# Autodesk Inventor assembly: CorpoInternoTurbinaAssemblato
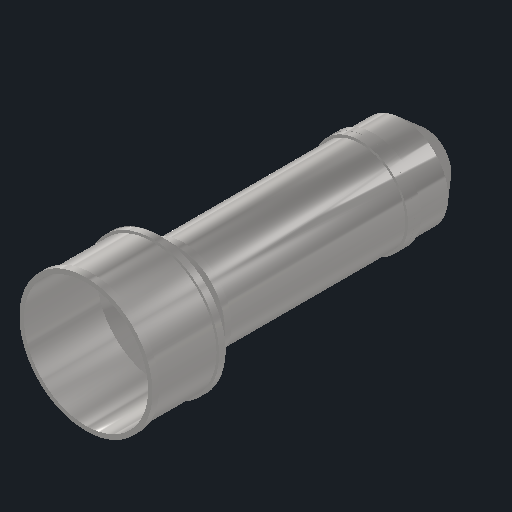
[picture p0: Inventor's stored thumbnail of the model, 512x512]
Saved by Autodesk Inventor 2026.2 (Build 302298010, 298A)
## iProperties
Created: 2026-05-01
Part Number: CorpoInternoTurbinaAssemblato
Document SubType Name: Assembly
Designer: Yan
Author: Yan
## Documents named in this file (5)
- C:\Users\Yan\Desktop\Turbina\CorpoInternoTurbinaAssemblato.iam
- C:\Users\Yan\Desktop\Turbina\CollegamentoCorpo1.ipt
- C:\Users\Yan\Desktop\Turbina\DiscoCorpoScarico.ipt
- C:\Users\Yan\Desktop\Turbina\DiscoCorpoTurbina2.ipt
- C:\Users\Yan\Desktop\Turbina\DiscoCorpoTurbina3.ipt
## Components (4 placed, 4 different names)
1. CollegamentoCorpo1:1 — Mate:1, Mate:2, Mate:4, Mate:5, Mate:6
2. DiscoCorpoScarico:1 — Mate:7, Mate:8
3. DiscoCorpoTurbina2:1 — Mate:1, Mate:3, Mate:4, Mate:6
4. DiscoCorpoTurbina3:1 — Mate:2, Mate:3, Mate:5, Mate:7, Mate:8
## Relationships (8: Mate 8)
- Mate:1: CollegamentoCorpo1:1 ↔ DiscoCorpoTurbina2:1
- Mate:2: CollegamentoCorpo1:1 ↔ DiscoCorpoTurbina3:1
- Mate:3: DiscoCorpoTurbina2:1 ↔ DiscoCorpoTurbina3:1
- Mate:4: CollegamentoCorpo1:1 ↔ DiscoCorpoTurbina2:1
- Mate:5: CollegamentoCorpo1:1 ↔ DiscoCorpoTurbina3:1
- Mate:6: CollegamentoCorpo1:1 ↔ DiscoCorpoTurbina2:1
- Mate:7: DiscoCorpoScarico:1 ↔ DiscoCorpoTurbina3:1
- Mate:8: DiscoCorpoScarico:1 ↔ DiscoCorpoTurbina3:1
